# Autodesk Inventor assembly: tower
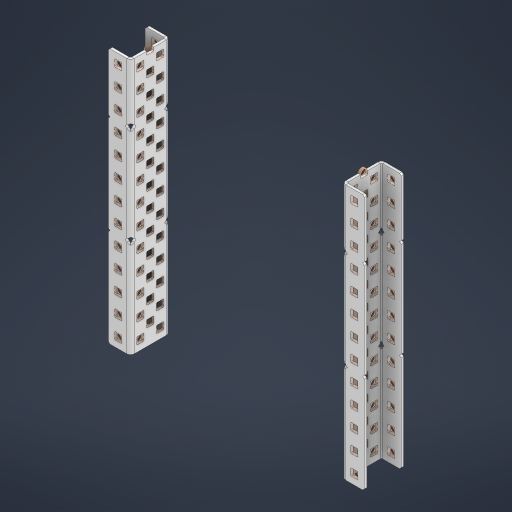
[picture p0: Inventor's stored thumbnail of the model, 512x512]
Saved by Autodesk Inventor 2024 (Build 280153000, 153)
## iProperties
Created: 2023-10-19
Part Number: tower
Document SubType Name: Assembly
Designer: avere
Author: avere
## Documents named in this file (2)
- C:\Users\avere\Documents\rbp_cad\goated_v0.1\catapult\tower.iam
- C:\Users\avere\Documents\rbp_cad\VEX-CAD-Inventor-1.41\Structure\C Channel\Aluminum 1x2x1\Alu C 1x2x1x13.ipt
## Components (3 placed, 1 different names)
1. Alu C 1x2x1x13:1 — Insert:1, Mate:1
2. Alu C 1x2x1x13:2 — Insert:2, Mate:2
3. Alu C 1x2x1x13:3 — Insert:1, Mate:1, Insert:2, Mate:2
## Relationships (4: Insert 2, Mate 2)
- Insert:1: Alu C 1x2x1x13:1 ↔ Alu C 1x2x1x13:3
- Mate:1: Alu C 1x2x1x13:1 ↔ Alu C 1x2x1x13:3
- Insert:2: Alu C 1x2x1x13:2 ↔ Alu C 1x2x1x13:3
- Mate:2: Alu C 1x2x1x13:2 ↔ Alu C 1x2x1x13:3
